# Autodesk Inventor assembly: Robot Dog lagi
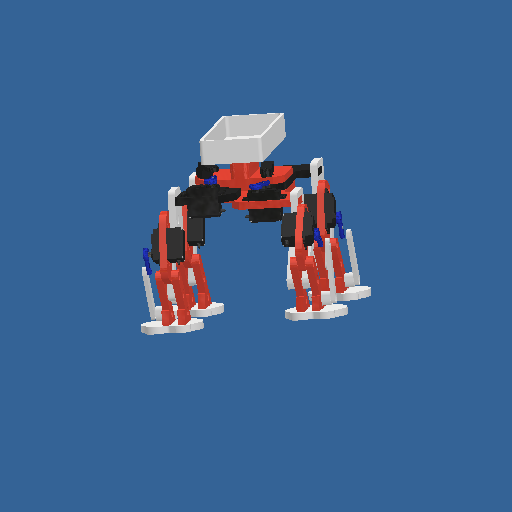
[picture p0: Inventor's stored thumbnail of the model, 512x512]
Saved by Autodesk Inventor 2027 (Build 310192000, 192)
## iProperties
Created: 2026-07-03
Part Number: Robot Dog lagi
Document SubType Name: Assembly
Designer: Martina
Author: Martina
## Documents named in this file (20)
- C:\Users\AL\Downloads\3d inventor\Robot Dog lagi.iam
- C:\Users\AL\Downloads\3d inventor\Hip.ipt
- C:\Users\AL\Downloads\3d inventor\KEPALA.ipt
- Kepala.ipt
- C:\Users\AL\Downloads\3d inventor\Leher Robot.ipt
- C:\Users\AL\Downloads\3d inventor\Atas Slider.ipt
- C:\Users\AL\Downloads\3d inventor\telapak kakii.ipt
- C:\Users\AL\Downloads\3d inventor\kaki tengah.ipt
- C:\Users\AL\Downloads\3d inventor\engsell.ipt
- engsel.ipt
- C:\Users\AL\Downloads\3d inventor\slider hitam.ipt
- slider hitam.ipt
- C:\Users\AL\Downloads\3d inventor\slider merah.ipt
- C:\Users\AL\Downloads\3d inventor\Spacer.ipt
- C:\Users\AL\Downloads\3d inventor\Uleg.ipt
- C:\Users\AL\Downloads\3d inventor\LegLverr.ipt
- C:\Users\AL\Downloads\3d inventor\arm servo.ipt
- C:\Users\AL\Downloads\3d inventor\Penggerak servo kanan.ipt
- C:\Users\AL\Downloads\3d inventor\Penggerak servo kiri.ipt
- C:\Users\AL\Downloads\3d inventor\Servoo0.iam
## Components (53 placed, 16 different names)
1. Kepala:1 — Mate:32, Mate:33, Mate:34
2. Leher Robot:1 — Mate:32, Mate:33, Mate:34, Mate:35, Mate:36, Mate:37
3. Atas Slider:1 — Mate:35, Mate:36, Mate:37, Flush:13, Mate:84, Rotational:30, Rotational:31, Mate:92
4. telapak kakii:1 — Mate:42, Flush:3, Mate:43, Mate:44, Flush:4, Mate:45
5. kaki tengah:1 — Mate:38, Flush:1, Mate:39, Rotational:2, Rotational:5, Rotational:9
6. telapak kakii:2 — Mate:38, Flush:1, Mate:39, Mate:40, Flush:2, Mate:41
7. kaki tengah:2 — Mate:40, Flush:2, Mate:41
8. kaki tengah:3 — Mate:42, Flush:3, Mate:43, Rotational:1, Rotational:12
9. kaki tengah:4 — Mate:44, Flush:4, Mate:45, Rotational:6, Rotational:11
10. engsel:1 — Rotational:1, Rotational:4, Mate:123, Mate:124, Mate:125
11. engsel:2 — Rotational:2, Rotational:3, Mate:129, Mate:130, Mate:131
12. Hip:4 — Mate:49, Flush:6, Mate:50, Rotational:4, Cylindrical:3, Cylindrical:4
13. Hip:5 — Mate:47, Flush:5, Mate:48, Rotational:3, Cylindrical:2
14. slider hitam:2 — Mate:47, Flush:5, Mate:48, Mate:49, Flush:6, Mate:50, Mate:83, Flush:13, Mate:84, Flush:14, Flush:15, Mate:132, Mate:133, Mate:134
15. slider merah:1 — Mate:83, Mate:92, Flush:14, Flush:15, Mate:104, Flush:20, Mate:105, Mate:116, Flush:23, Mate:117, Mate:135, Mate:136, Mate:137
16. Spacer:1 — Rotational:6, Rotational:7
17. Spacer:2 — Rotational:5, Rotational:8
18. Uleg:1 — Rotational:7, Cylindrical:5
19. Uleg:2 — Rotational:8, Rotational:14
20. LegLverr:1 — Rotational:9, Cylindrical:2
21. LegLverr:2 — Rotational:11, Cylindrical:4
22. LegLverr:4 — Rotational:12, Cylindrical:3
23. arm servo:1 — Cylindrical:5, Cylindrical:23
24. arm servo:2 — Rotational:14, Cylindrical:25
25. Penggerak servo kanan:1 — Rotational:30, Cylindrical:16
26. Penggerak servo kiri:1 — Rotational:31, Cylindrical:15
27. arm servo:5 — Cylindrical:15, Cylindrical:26
28. arm servo:6 — Cylindrical:16, Cylindrical:27
29. telapak kakii:5
30. kaki tengah:11
31. kaki tengah:12
32. engsel:5 — Mate:126, Mate:127, Mate:128
33. Hip:8 — Mate:104, Flush:20, Mate:105
34. Spacer:5
35. Uleg:5
36. LegLverr:10
37. LegLverr:11
38. arm servo:7 — Cylindrical:24
39. kaki tengah:13
40. telapak kakii:6
41. kaki tengah:14
42. engsel:6 — Mate:120, Mate:121, Mate:122
43. Hip:9 — Mate:116, Flush:23, Mate:117
44. Spacer:6
45. Uleg:6
46. LegLverr:12
47. arm servo:8 — Cylindrical:22
48. Servoo0:1 [sub-assembly] — Mate:120, Mate:121, Mate:122, Cylindrical:22
49. Servoo0:2 [sub-assembly] — Mate:123, Mate:124, Mate:125, Cylindrical:23
50. Servoo0:3 [sub-assembly] — Mate:126, Mate:127, Mate:128, Cylindrical:24
51. Servoo0:4 [sub-assembly] — Mate:129, Mate:130, Mate:131, Cylindrical:25
52. Servoo0:5 [sub-assembly] — Mate:132, Mate:133, Mate:134, Cylindrical:26
53. Servoo0:6 [sub-assembly] — Mate:135, Mate:136, Mate:137, Cylindrical:27
## Relationships (108: Mate 51, RevoluteJoint 26, CylindricalJoint 16, Flush 15)
- Mate:32: Kepala:1 ↔ Leher Robot:1
- Mate:33: Kepala:1 ↔ Leher Robot:1
- Mate:34: Kepala:1 ↔ Leher Robot:1
- Mate:35: Leher Robot:1 ↔ Atas Slider:1
- Mate:36: Leher Robot:1 ↔ Atas Slider:1
- Mate:37: Leher Robot:1 ↔ Atas Slider:1
- Mate:38: kaki tengah:1 ↔ telapak kakii:2
- Flush:1: kaki tengah:1 ↔ telapak kakii:2
- Mate:39: kaki tengah:1 ↔ telapak kakii:2
- Mate:40: telapak kakii:2 ↔ kaki tengah:2
- Flush:2: telapak kakii:2 ↔ kaki tengah:2
- Mate:41: telapak kakii:2 ↔ kaki tengah:2
- Mate:42: telapak kakii:1 ↔ kaki tengah:3
- Flush:3: telapak kakii:1 ↔ kaki tengah:3
- Mate:43: telapak kakii:1 ↔ kaki tengah:3
- Mate:44: telapak kakii:1 ↔ kaki tengah:4
- Flush:4: telapak kakii:1 ↔ kaki tengah:4
- Mate:45: telapak kakii:1 ↔ kaki tengah:4
- Rotational:1 [RevoluteJoint] (-1 mm): kaki tengah:3 ↔ engsel:1
- Rotational:2 [RevoluteJoint] (-1 mm): kaki tengah:1 ↔ engsel:2
- Mate:47: Hip:5 ↔ slider hitam:2
- Flush:5: Hip:5 ↔ slider hitam:2
- Mate:48: Hip:5 ↔ slider hitam:2
- Mate:49: Hip:4 ↔ slider hitam:2
- Flush:6: Hip:4 ↔ slider hitam:2
- Mate:50: Hip:4 ↔ slider hitam:2
- Rotational:3 [RevoluteJoint] (-1 mm): engsel:2 ↔ Hip:5
- Rotational:4 [RevoluteJoint] (1 mm): engsel:1 ↔ Hip:4
- Rotational:5 [RevoluteJoint]: kaki tengah:1 ↔ Spacer:2
- Rotational:6 [RevoluteJoint]: kaki tengah:4 ↔ Spacer:1
- Rotational:7 [RevoluteJoint] (1 mm): Spacer:1 ↔ Uleg:1
- Rotational:8 [RevoluteJoint] (1 mm): Spacer:2 ↔ Uleg:2
- Rotational:9 [RevoluteJoint] (-1 mm): kaki tengah:1 ↔ LegLverr:1
- Rotational:11 [RevoluteJoint] (-1 mm): kaki tengah:4 ↔ LegLverr:2
- Rotational:12 [RevoluteJoint]: kaki tengah:3 ↔ LegLverr:4
- Cylindrical:2: Hip:5 ↔ LegLverr:1
- Cylindrical:3: Hip:4 ↔ LegLverr:4
- Cylindrical:4: Hip:4 ↔ LegLverr:2
- Cylindrical:5: Uleg:1 ↔ arm servo:1
- Rotational:14 [RevoluteJoint]: Uleg:2 ↔ arm servo:2
- Mate:83: slider hitam:2 ↔ slider merah:1
- Flush:13: Atas Slider:1 ↔ slider hitam:2
- Mate:84: Atas Slider:1 ↔ slider hitam:2
- Rotational:30 [RevoluteJoint]: Atas Slider:1 ↔ Penggerak servo kanan:1
- Rotational:31 [RevoluteJoint]: Atas Slider:1 ↔ Penggerak servo kiri:1
- Mate:92: Atas Slider:1 ↔ slider merah:1
- Flush:14: slider hitam:2 ↔ slider merah:1
- Flush:15: slider hitam:2 ↔ slider merah:1
- Cylindrical:15: Penggerak servo kiri:1 ↔ arm servo:5
- Cylindrical:16: Penggerak servo kanan:1 ↔ arm servo:6
- [Mate]: telapak kakii:5 ↔ kaki tengah:11
- [Flush]: telapak kakii:5 ↔ kaki tengah:11
- [Mate]: telapak kakii:5 ↔ kaki tengah:11
- [Mate]: telapak kakii:5 ↔ kaki tengah:12
- [Flush]: telapak kakii:5 ↔ kaki tengah:12
- [Mate]: telapak kakii:5 ↔ kaki tengah:12
- [RevoluteJoint] (-1 mm): kaki tengah:11 ↔ engsel:5
- [RevoluteJoint] (1 mm): engsel:5 ↔ Hip:8
- [RevoluteJoint]: kaki tengah:12 ↔ Spacer:5
- [RevoluteJoint] (1 mm): Spacer:5 ↔ Uleg:5
- [RevoluteJoint] (-1 mm): kaki tengah:12 ↔ LegLverr:10
- [RevoluteJoint]: kaki tengah:11 ↔ LegLverr:11
- [CylindricalJoint]: Hip:8 ↔ LegLverr:11
- [CylindricalJoint]: Hip:8 ↔ LegLverr:10
- [CylindricalJoint]: Uleg:5 ↔ arm servo:7
- Mate:104: slider merah:1 ↔ Hip:8
- Flush:20: slider merah:1 ↔ Hip:8
- Mate:105: slider merah:1 ↔ Hip:8
- [Mate]: kaki tengah:13 ↔ telapak kakii:6
- [Flush]: kaki tengah:13 ↔ telapak kakii:6
- [Mate]: kaki tengah:13 ↔ telapak kakii:6
- [Mate]: telapak kakii:6 ↔ kaki tengah:14
- [Flush]: telapak kakii:6 ↔ kaki tengah:14
- [Mate]: telapak kakii:6 ↔ kaki tengah:14
- [RevoluteJoint] (-1 mm): kaki tengah:13 ↔ engsel:6
- [RevoluteJoint] (-1 mm): engsel:6 ↔ Hip:9
- [RevoluteJoint]: kaki tengah:13 ↔ Spacer:6
- [RevoluteJoint] (1 mm): Spacer:6 ↔ Uleg:6
- [RevoluteJoint] (-1 mm): kaki tengah:13 ↔ LegLverr:12
- [CylindricalJoint]: Hip:9 ↔ LegLverr:12
- [RevoluteJoint]: Uleg:6 ↔ arm servo:8
- Mate:116: slider merah:1 ↔ Hip:9
- Flush:23: slider merah:1 ↔ Hip:9
- Mate:117: slider merah:1 ↔ Hip:9
- Mate:120: engsel:6 ↔ Servoo0:1
- Mate:121: engsel:6 ↔ Servoo0:1
- Mate:122: engsel:6 ↔ Servoo0:1
- Cylindrical:22: arm servo:8 ↔ Servoo0:1
- Mate:123: engsel:1 ↔ Servoo0:2
- Mate:124: engsel:1 ↔ Servoo0:2
- Mate:125: engsel:1 ↔ Servoo0:2
- Cylindrical:23: arm servo:1 ↔ Servoo0:2
- Mate:126: engsel:5 ↔ Servoo0:3
- Mate:127: engsel:5 ↔ Servoo0:3
- Mate:128: engsel:5 ↔ Servoo0:3
- Cylindrical:24: arm servo:7 ↔ Servoo0:3
- Mate:129: engsel:2 ↔ Servoo0:4
- Mate:130: engsel:2 ↔ Servoo0:4
- Mate:131: engsel:2 ↔ Servoo0:4
- Cylindrical:25: arm servo:2 ↔ Servoo0:4
- Mate:132: slider hitam:2 ↔ Servoo0:5
- Mate:133: slider hitam:2 ↔ Servoo0:5
- Mate:134: slider hitam:2 ↔ Servoo0:5
- Cylindrical:26: arm servo:5 ↔ Servoo0:5
- Mate:135: slider merah:1 ↔ Servoo0:6
- Mate:136: slider merah:1 ↔ Servoo0:6
- Mate:137: slider merah:1 ↔ Servoo0:6
- Cylindrical:27: arm servo:6 ↔ Servoo0:6
## Named parameters: d286_d164 = 40.265945 deg, d287_d165 = 0 mm, d288_d166 = -49.734055 deg, d289_d167 = 9.8 mm, d295_d173 = 133.443275 deg, d296_d174 = -3.46307 mm, d299_d142 = 0 mm, d300_d143 = -137.52327 deg, d301_d144 = 1 mm, d302_d145 = -166.686345 deg, d307_d156 = -1 mm, d308_d157 = 42.171796 deg, d309_d158 = 0 mm, d310_d159 = -137.828204 deg, d311_d84 = 0 mm, d312_d85 = 0 mm, d313_d86 = 0 mm, d314_d87 = 0 mm, d315_d88 = -1 mm, d316_d89 = 2.890078 deg, d317_d114 = 1 mm, d318_d115 = 130.204072 deg, d325_d82 = 0 mm, d326_d83 = 0 mm, d340_d162 = 26.322627 deg, d341_d163 = 1 mm, d348_d181 = 0 mm, d349_d182 = 79.377218 deg, d350_d140 = 0 mm, d351_d141 = 111.282941 deg, d352_d146 = 1 mm, d353_d147 = -147.231599 deg, d354_d152 = -1 mm, d355_d153 = 159.300561 deg, d356_d90 = -1 mm, d357_d91 = 23.963333 deg, d361_d112 = -1 mm, d362_d113 = 64.014602 deg, d363_d76 = 0 mm, d364_d77 = 0 mm, d365_d78 = 0 mm, d366_d79 = 0 mm, d367_d80 = 0 mm, d368_d81 = 0 mm
